# Autodesk Inventor assembly: Hektor3D
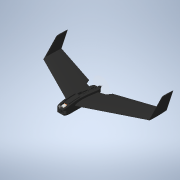
[picture p0: Inventor's stored thumbnail of the model, 180x180]
Saved by Autodesk Inventor 2020 (Build 240168000, 168)
## iProperties
Part Number: Hektor3D
Document SubType Name: Assembly
Designer: Admin
Mass: 21163.6 g
Surface Area: 21673.8 cm^2
Volume: 18590.6 cm^3
Density: 1.1384 g/cm^3
Revision: -
VAULT_Status: in Bearbeitung
Gewicht: 21,164 kg
InventorVersion: 2019.4
Author: Admin
## Documents named in this file (20)
- C:\Users\MartinDJay\Documents\GitHub\CAD_Elements\CAD\Hektor\Hektor_3D\Hektor3D.iam
- HEKTOR3D_HEKTOR3D.IAM
- C:\Users\MartinDJay\Documents\GitHub\CAD_Elements\CAD\Hektor\Hektor_3D\Rumpfhälfte.ipt
- C:\Users\MartinDJay\Documents\GitHub\CAD_Elements\CAD\Hektor\Hektor_3D\Rumpfhälfte1.ipt
- C:\Users\MartinDJay\Documents\GitHub\CAD_Elements\CAD\Hektor\Hektor_3D\wing_r.ipt
- C:\Users\MartinDJay\Documents\GitHub\CAD_Elements\CAD\Hektor\Hektor_3D\Wing_L.ipt
- C:\Users\MartinDJay\Documents\GitHub\CAD_Elements\CAD\Hektor\Hektor_3D\Winlet_R.ipt
- C:\Users\MartinDJay\Documents\GitHub\CAD_Elements\CAD\Hektor\Hektor_3D\Winglet_L.ipt
- C:\Users\MartinDJay\Documents\GitHub\CAD_Elements\CAD\Hektor\Hektor_3D\canopy.ipt
- C:\Users\MartinDJay\Documents\GitHub\CAD_Elements\Hilfsdateien\Gopro Hero 6-7.ipt
- C:\Users\MartinDJay\Documents\GitHub\CAD_Elements\CAD\Hektor\Airunit_aufnahme.ipt
- C:\Users\MartinDJay\Documents\GitHub\CAD_Elements\Hilfsdateien\Runcam5.ipt
- C:\Users\MartinDJay\Documents\GitHub\CAD_Elements\Hilfsdateien\DJI FPV Air Unit.ipt
- C:\Users\MartinDJay\Documents\GitHub\CAD_Elements\Hilfsdateien\DJI FPV Camera.ipt
- C:\Users\MartinDJay\Documents\GitHub\CAD_Elements\Hilfsdateien\DJIAirUnit_Mount_v1.ipt
- C:\Users\MartinDJay\Documents\GitHub\CAD_Elements\Hilfsdateien\4S5000.ipt
- C:\Users\MartinDJay\Documents\GitHub\CAD_Elements\CAD\Hektor\Hektor_3D\Props.ipt
- C:\Users\MartinDJay\Documents\GitHub\CAD_Elements\CAD\Motor\CobraCP2814-1050kv.ipt
- C:\Users\MartinDJay\Documents\GitHub\CAD_Elements\Hilfsdateien\GoPro9.ipt
- C:\Users\MartinDJay\Documents\GitHub\CAD_Elements\Hilfsdateien\DJI FPV Air Unit.STEP
## Components (17 placed, 17 different names)
1. RUMPFHÄLFTE_RUMPFHÄLFTE:1 — Fluchtend:1, Fluchtend:2, Fluchtend:3, Passend:3, Passend:4, Passend:23, Winkel:4, Passend:59, Passend:63, Passend:64, Passend:74, Passend:78, Passend:82
2. RUMPFHÄLFTE1_RUMPFHÄLFTE1:1 — Passend:1, Fluchtend:4, Passend:2, Passend:5, Passend:6, Passend:24, Passend:40, Passend:70, Passend:72
3. WING_R_WING_R:1 — Passend:3, Passend:4, Passend:9, Fluchtend:12, Passend:38, Winkel:4, Passend:39
4. WING_L_WING_L:1 — Passend:5, Passend:6, Passend:12, Passend:38
5. WINLET_R_WINLET_R:1 — Passend:9, Fluchtend:12, Fluchtend:13, Passend:11, Passend:39
6. WINGLET_L_WINGLET_L:1 — Fluchtend:13, Passend:11, Passend:12
7. CANOPY_CANOPY:1 — Passend:23, Passend:24, Fluchtend:15, Passend:40
8. AIRUNIT_AUFNAHME_AIRUNIT_AUFNAHME--IPT:1 — Passend:74, Passend:77, Passend:78, Passend:79, Passend:80, Passend:81, Passend:82
9. DJIAIRUNIT_MOUNT_V1_DJIAIRUNIT_MOUNT_V1--IPT:1 — Passend:65, Passend:66, Passend:67, Passend:77
10. 4S5000:1 — Passend:62, Passend:63, Passend:64
11. PROPS_PROPS--IPT:1 — Passend:57, Passend:58
12. COBRACP2814-1050KV_COBRACP2814-1050KV--IPT:1 — Passend:57, Passend:58, Passend:59, Passend:60, Passend:61, Winkel:5
13. Gopro Hero 6-7:1 — Fluchtend:45, Fluchtend:46, Passend:70, Passend:72
14. GoPro9:1 — Fluchtend:45, Fluchtend:46
15. DJI FPV Air Unit:1 — Passend:65, Passend:66, Passend:67
16. DJI FPV Camera:1 — Passend:79, Passend:80, Passend:81
17. Runcam5:1
## Relationships (45: Mate 34, Flush 9, Angle 2)
- Fluchtend:1 [Flush] (2 mm): RUMPFHÄLFTE_RUMPFHÄLFTE:1
- Fluchtend:2 [Flush]: RUMPFHÄLFTE_RUMPFHÄLFTE:1
- Fluchtend:3 [Flush] (75 mm): RUMPFHÄLFTE_RUMPFHÄLFTE:1
- Passend:1 [Mate] (-75 mm): RUMPFHÄLFTE1_RUMPFHÄLFTE1:1
- Fluchtend:4 [Flush]: RUMPFHÄLFTE1_RUMPFHÄLFTE1:1
- Passend:2 [Mate] (2 mm): RUMPFHÄLFTE1_RUMPFHÄLFTE1:1
- Passend:3 [Mate]: RUMPFHÄLFTE_RUMPFHÄLFTE:1 ↔ WING_R_WING_R:1
- Passend:4 [Mate]: RUMPFHÄLFTE_RUMPFHÄLFTE:1 ↔ WING_R_WING_R:1
- Passend:5 [Mate]: RUMPFHÄLFTE1_RUMPFHÄLFTE1:1 ↔ WING_L_WING_L:1
- Passend:6 [Mate]: RUMPFHÄLFTE1_RUMPFHÄLFTE1:1 ↔ WING_L_WING_L:1
- Passend:9 [Mate] (-12 mm): WING_R_WING_R:1 ↔ WINLET_R_WINLET_R:1
- Fluchtend:12 [Flush] (340 mm): WING_R_WING_R:1 ↔ WINLET_R_WINLET_R:1
- Fluchtend:13 [Flush]: WINLET_R_WINLET_R:1 ↔ WINGLET_L_WINGLET_L:1
- Passend:11 [Mate]: WINLET_R_WINLET_R:1 ↔ WINGLET_L_WINGLET_L:1
- Passend:12 [Mate]: WING_L_WING_L:1 ↔ WINGLET_L_WINGLET_L:1
- Passend:23 [Mate]: RUMPFHÄLFTE_RUMPFHÄLFTE:1 ↔ CANOPY_CANOPY:1
- Passend:24 [Mate] (2 mm): RUMPFHÄLFTE1_RUMPFHÄLFTE1:1 ↔ CANOPY_CANOPY:1
- Fluchtend:15 [Flush]: CANOPY_CANOPY:1
- Passend:38 [Mate]: WING_R_WING_R:1 ↔ WING_L_WING_L:1
- Winkel:4 [Angle] (180 deg): RUMPFHÄLFTE_RUMPFHÄLFTE:1 ↔ WING_R_WING_R:1
- Passend:39 [Mate]: WING_R_WING_R:1 ↔ WINLET_R_WINLET_R:1
- Passend:40 [Mate]: RUMPFHÄLFTE1_RUMPFHÄLFTE1:1 ↔ CANOPY_CANOPY:1
- Passend:57 [Mate]: PROPS_PROPS--IPT:1 ↔ COBRACP2814-1050KV_COBRACP2814-1050KV--IPT:1
- Passend:58 [Mate] (4 mm): PROPS_PROPS--IPT:1 ↔ COBRACP2814-1050KV_COBRACP2814-1050KV--IPT:1
- Passend:59 [Mate]: RUMPFHÄLFTE_RUMPFHÄLFTE:1 ↔ COBRACP2814-1050KV_COBRACP2814-1050KV--IPT:1
- Passend:60 [Mate]: COBRACP2814-1050KV_COBRACP2814-1050KV--IPT:1
- Passend:61 [Mate] (-8 mm): COBRACP2814-1050KV_COBRACP2814-1050KV--IPT:1
- Winkel:5 [Angle] (45 deg): COBRACP2814-1050KV_COBRACP2814-1050KV--IPT:1
- Passend:62 [Mate]: 4S5000:1
- Passend:63 [Mate] (2 mm): RUMPFHÄLFTE_RUMPFHÄLFTE:1 ↔ 4S5000:1
- Passend:64 [Mate] (5 mm): RUMPFHÄLFTE_RUMPFHÄLFTE:1 ↔ 4S5000:1
- Fluchtend:45 [Flush]: Gopro Hero 6-7:1 ↔ GoPro9:1
- Fluchtend:46 [Flush]: Gopro Hero 6-7:1 ↔ GoPro9:1
- Passend:65 [Mate]: DJIAIRUNIT_MOUNT_V1_DJIAIRUNIT_MOUNT_V1--IPT:1 ↔ DJI FPV Air Unit:1
- Passend:66 [Mate]: DJIAIRUNIT_MOUNT_V1_DJIAIRUNIT_MOUNT_V1--IPT:1 ↔ DJI FPV Air Unit:1
- Passend:67 [Mate]: DJIAIRUNIT_MOUNT_V1_DJIAIRUNIT_MOUNT_V1--IPT:1 ↔ DJI FPV Air Unit:1
- Passend:70 [Mate]: RUMPFHÄLFTE1_RUMPFHÄLFTE1:1 ↔ Gopro Hero 6-7:1
- Passend:72 [Mate] (0.25 mm): RUMPFHÄLFTE1_RUMPFHÄLFTE1:1 ↔ Gopro Hero 6-7:1
- Passend:74 [Mate]: RUMPFHÄLFTE_RUMPFHÄLFTE:1 ↔ AIRUNIT_AUFNAHME_AIRUNIT_AUFNAHME--IPT:1
- Passend:77 [Mate]: AIRUNIT_AUFNAHME_AIRUNIT_AUFNAHME--IPT:1 ↔ DJIAIRUNIT_MOUNT_V1_DJIAIRUNIT_MOUNT_V1--IPT:1
- Passend:78 [Mate]: RUMPFHÄLFTE_RUMPFHÄLFTE:1 ↔ AIRUNIT_AUFNAHME_AIRUNIT_AUFNAHME--IPT:1
- Passend:79 [Mate] (0.25 mm): AIRUNIT_AUFNAHME_AIRUNIT_AUFNAHME--IPT:1 ↔ DJI FPV Camera:1
- Passend:80 [Mate] (0.25 mm): AIRUNIT_AUFNAHME_AIRUNIT_AUFNAHME--IPT:1 ↔ DJI FPV Camera:1
- Passend:81 [Mate]: AIRUNIT_AUFNAHME_AIRUNIT_AUFNAHME--IPT:1 ↔ DJI FPV Camera:1
- Passend:82 [Mate]: RUMPFHÄLFTE_RUMPFHÄLFTE:1 ↔ AIRUNIT_AUFNAHME_AIRUNIT_AUFNAHME--IPT:1
## Named parameters: Gewicht = 21.1636
note: some values were not read from the file. Shown as the stored number, unit unknown: "Gewicht".
